# Autodesk Inventor assembly: GlassesAssembly
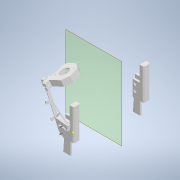
[picture p0: Inventor's stored thumbnail of the model, 180x180]
Saved by Autodesk Inventor 2020 (Build 240168000, 168)
## iProperties
Created: 2020-03-20
Part Number: GlassesAssembly
Document SubType Name: Assembly
Designer: Fynn
Author: Fynn
## Documents named in this file (10)
- I:\Daten\PA\Neues Thema\CADFiles\Neuer Ordner\GlassesAssembly.iam
- I:\Daten\PA\Neues Thema\CADFiles\Neuer Ordner\Brillenbuegel.ipt
- I:\Daten\PA\Neues Thema\CADFiles\Neuer Ordner\CemaraArmInterface.ipt
- C:\Users\Fynn\Documents\Inventor\Content Center Files\R2020\de-DE\ISO 4762(1)\DIN EN ISO 4762 - M2 x 20.ipt
- I:\Daten\PA\Neues Thema\CADFiles\Neuer Ordner\CameraArm.ipt
- I:\Daten\PA\Neues Thema\CADFiles\Neuer Ordner\BallJoint.ipt
- I:\Daten\PA\Neues Thema\CADFiles\Neuer Ordner\BallJointClamp.ipt
- I:\Daten\PA\Neues Thema\CADFiles\Neuer Ordner\Brillenbuegel_MIR.ipt
- I:\Daten\PA\Neues Thema\CADFiles\Neuer Ordner\CemaraArmInterface_MIR.ipt
- I:\Daten\PA\Neues Thema\CADFiles\Neuer Ordner\CameraMoldLogi.ipt
## Components (10 placed, 9 different names)
1. Brillenbuegel:1 — Passend:1, Passend:2, Fluchtend:1, Passend:3, Passend:4, Passend:5, Passend:6, Passend:8
2. CemaraArmInterface:1 — Passend:3, Passend:4, Passend:5, Passend:7, Passend:9, Fluchtend:2, Passend:11
3. DIN EN ISO 4762 M2 x 20:1 — Passend:6, Passend:7
4. DIN EN ISO 4762 M2 x 20:2 — Passend:8, Passend:9, Passend:10
5. CameraArm:1 — Fluchtend:2, Fluchtend:3, Fluchtend:4, Fluchtend:5, Passend:10, Passend:11
6. BallJoint:1 — Fluchtend:3, Fluchtend:4, Fluchtend:5, Tangential:1, Tangential:2
7. BallJointClamp:1 — Passend:15, Passend:16, Tangential:2
8. Brillenbuegel_MIR:1 — Passend:12, Passend:13, Passend:14
9. CemaraArmInterface_MIR:1
10. CameraMoldLogi:1 — Tangential:1, Passend:15, Passend:16
## Relationships (24: Mate 16, Flush 6, Tangent 2)
- Passend:1 [Mate]: Brillenbuegel:1
- Passend:2 [Mate]: Brillenbuegel:1
- Fluchtend:1 [Flush]: Brillenbuegel:1
- Passend:3 [Mate]: Brillenbuegel:1 ↔ CemaraArmInterface:1
- Passend:4 [Mate]: Brillenbuegel:1 ↔ CemaraArmInterface:1
- Passend:5 [Mate] (0.5 mm): Brillenbuegel:1 ↔ CemaraArmInterface:1
- Passend:6 [Mate]: Brillenbuegel:1 ↔ DIN EN ISO 4762 M2 x 20:1
- Passend:7 [Mate]: CemaraArmInterface:1 ↔ DIN EN ISO 4762 M2 x 20:1
- Passend:8 [Mate]: Brillenbuegel:1 ↔ DIN EN ISO 4762 M2 x 20:2
- Passend:9 [Mate]: CemaraArmInterface:1 ↔ DIN EN ISO 4762 M2 x 20:2
- Fluchtend:2 [Flush]: CemaraArmInterface:1 ↔ CameraArm:1
- Fluchtend:3 [Flush]: CameraArm:1 ↔ BallJoint:1
- Fluchtend:4 [Flush]: CameraArm:1 ↔ BallJoint:1
- Fluchtend:5 [Flush]: CameraArm:1 ↔ BallJoint:1
- Passend:10 [Mate]: DIN EN ISO 4762 M2 x 20:2 ↔ CameraArm:1
- Passend:11 [Mate]: CemaraArmInterface:1 ↔ CameraArm:1
- Fluchtend:8 [Flush] (65 mm)
- Passend:12 [Mate]: Brillenbuegel_MIR:1
- Passend:13 [Mate]: Brillenbuegel_MIR:1
- Passend:14 [Mate]: Brillenbuegel_MIR:1
- Tangential:1: BallJoint:1 ↔ CameraMoldLogi:1
- Passend:15 [Mate]: BallJointClamp:1 ↔ CameraMoldLogi:1
- Passend:16 [Mate]: BallJointClamp:1 ↔ CameraMoldLogi:1
- Tangential:2: BallJoint:1 ↔ BallJointClamp:1
